# Autodesk Inventor assembly: wheel
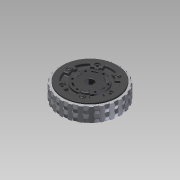
[picture p0: Inventor's stored thumbnail of the model, 180x180]
Saved by Autodesk Inventor 2015 (Build 190159000, 159)
## iProperties
Created: 2015-12-17
Part Number: wheel
Document SubType Name: Assembly
Designer: Daniel
Author: Daniel
## Documents named in this file (4)
- C:\Users\Daniel\Documents\inventor\West Coast Drive\wheel.iam
- C:\Users\Daniel\Documents\inventor\West Coast Drive\217-2588 wheel hub.iam
- C:\Users\Daniel\Documents\inventor\West Coast Drive\217-2859 tire tread.iam
- C:\Users\Daniel\Documents\inventor\West Coast Drive\217-4009- plastic hex hub.ipt
## Components (5 placed, 3 different names)
1. 217-2588 wheel hub:1 [sub-assembly] — Mate:1, Mate:2, Mate:5, Mate:6, Mate:7, Mate:8, Mate:9, Mate:10, Mate:11
2. 217-2859 tire tread:1 [sub-assembly] — Mate:1, Mate:3, Mate:4
3. 217-2859 tire tread:2 [sub-assembly] — Mate:2, Mate:3, Mate:4, Mate:5
4. 217-4009- plastic hex hub:1 — Mate:9, Mate:10, Mate:11
5. 217-4009- plastic hex hub:2 — Mate:6, Mate:7, Mate:8
## Relationships (11: Mate 11)
- Mate:1: 217-2588 wheel hub:1 ↔ 217-2859 tire tread:1
- Mate:2: 217-2588 wheel hub:1 ↔ 217-2859 tire tread:2
- Mate:3: 217-2859 tire tread:1 ↔ 217-2859 tire tread:2
- Mate:4: 217-2859 tire tread:1 ↔ 217-2859 tire tread:2
- Mate:5: 217-2588 wheel hub:1 ↔ 217-2859 tire tread:2
- Mate:6: 217-2588 wheel hub:1 ↔ 217-4009- plastic hex hub:2
- Mate:7: 217-2588 wheel hub:1 ↔ 217-4009- plastic hex hub:2
- Mate:8: 217-2588 wheel hub:1 ↔ 217-4009- plastic hex hub:2
- Mate:9: 217-2588 wheel hub:1 ↔ 217-4009- plastic hex hub:1
- Mate:10: 217-2588 wheel hub:1 ↔ 217-4009- plastic hex hub:1
- Mate:11: 217-2588 wheel hub:1 ↔ 217-4009- plastic hex hub:1
